# Autodesk Inventor assembly: Circuito_Electrico
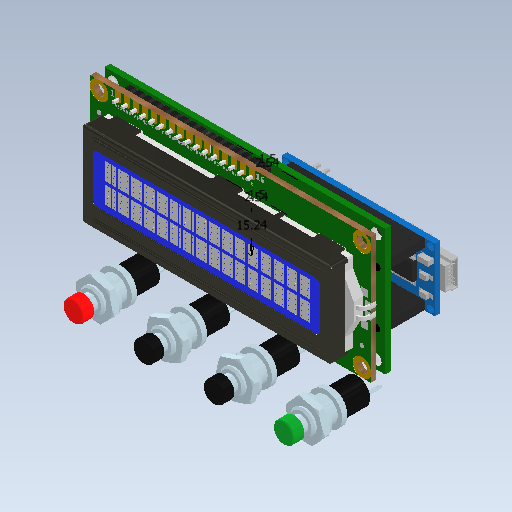
[picture p0: Inventor's stored thumbnail of the model, 512x512]
Saved by Autodesk Inventor 2020.1 (Build 241239000, 239)
## iProperties
Created: 2019-12-09
Part Number: Circuito_Electrico
Document SubType Name: Assembly
Designer: Daniel
Author: Daniel
## Documents named in this file (7)
- F:\Proyectos\Dog Feeder\Solido\Circuito Electrico\Circuito_Electrico.iam
- F:\Proyectos\Dog Feeder\Solido\Circuito Electrico\1602 LCD.ipt
- F:\Proyectos\Dog Feeder\Solido\Circuito Electrico\PCB.ipt
- F:\Proyectos\Dog Feeder\Solido\Circuito Electrico\Arduino y headers\Arduino NanoV3 + Female Headers.iam
- F:\Proyectos\Dog Feeder\Solido\Circuito Electrico\PushButton\SPST-NO.iam
- F:\Proyectos\Dog Feeder\Solido\Circuito Electrico\PushButton\SPST-NO Rojo.iam
- F:\Proyectos\Dog Feeder\Solido\Circuito Electrico\PushButton\SPST-NO Verde.iam
## Components (7 placed, 6 different names)
1. 1602 LCD:1 — Mate:1, Mate:2, Mate:3, Flush:2, Flush:3
2. PCB:1 — Mate:1, Mate:2, Mate:3, Mate:4, Mate:5, Flush:1, Mate:9, Mate:10, Mate:11, Mate:12
3. Arduino NanoV3 + Female Headers:1 [sub-assembly] — Mate:4, Mate:5, Flush:1
4. SPST-NO Rojo:1 [sub-assembly] — Mate:6, Mate:9, Flush:5, Symmetry:1
5. SPST-NO:2 [sub-assembly] — Mate:7, Mate:8, Mate:11, Flush:3, Flush:4
6. SPST-NO:3 [sub-assembly] — Mate:6, Mate:7, Mate:10, Flush:4, Flush:5
7. SPST-NO Verde:1 [sub-assembly] — Mate:8, Mate:12, Flush:2, Symmetry:1
## Relationships (18: Mate 12, Flush 5, Symmetry 1)
- Mate:1: 1602 LCD:1 ↔ PCB:1
- Mate:2: 1602 LCD:1 ↔ PCB:1
- Mate:3: 1602 LCD:1 ↔ PCB:1
- Mate:4: PCB:1 ↔ Arduino NanoV3 + Female Headers:1
- Mate:5: PCB:1 ↔ Arduino NanoV3 + Female Headers:1
- Flush:1 (-3 mm): PCB:1 ↔ Arduino NanoV3 + Female Headers:1
- Mate:6 (20 mm): SPST-NO Rojo:1 ↔ SPST-NO:3
- Mate:7 (20 mm): SPST-NO:2 ↔ SPST-NO:3
- Mate:8 (20 mm): SPST-NO:2 ↔ SPST-NO Verde:1
- Mate:9 (10 mm): PCB:1 ↔ SPST-NO Rojo:1
- Mate:10 (10 mm): PCB:1 ↔ SPST-NO:3
- Mate:11 (10 mm): PCB:1 ↔ SPST-NO:2
- Mate:12 (10 mm): PCB:1 ↔ SPST-NO Verde:1
- Flush:2: 1602 LCD:1 ↔ SPST-NO Verde:1
- Flush:3: 1602 LCD:1 ↔ SPST-NO:2
- Flush:4: SPST-NO:2 ↔ SPST-NO:3
- Flush:5: SPST-NO Rojo:1 ↔ SPST-NO:3
- Symmetry:1: SPST-NO Rojo:1 ↔ SPST-NO Verde:1
